# Autodesk Inventor assembly: linkage_system_test
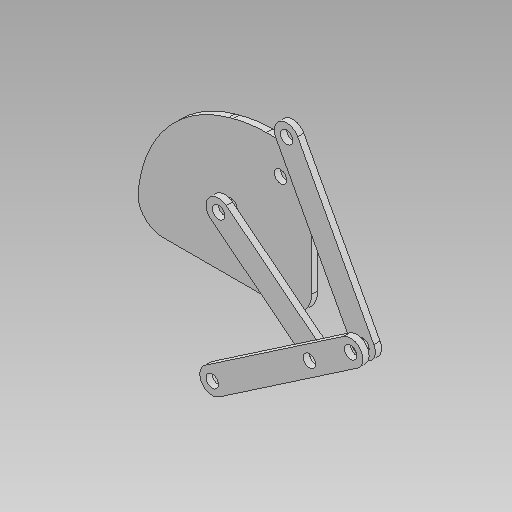
[picture p0: Inventor's stored thumbnail of the model, 512x512]
Saved by Autodesk Inventor 2025 (Build 290162000, 162)
## iProperties
Created: 2024-09-22
Part Number: linkage_system_test
Document SubType Name: Assembly
Designer: OSB
Title: S500 Frame
Author: OSB
Sending System: Autodesk Inventor 2021
Preprocessor: unknown
Minimum Resolution: 0.01
Sent Units: Millimeter
Translation Standard: IGES 5.3
Model Creation Time: 2020-07-07
## Documents named in this file (5)
- C:\Users\OSB\Desktop\SB\1.Projects\4_2\캡스톤 디자인(2)\linkage_system_test.iam
- C:\Users\OSB\Desktop\SB\1.Projects\4_2\캡스톤 디자인(2)\link_l1.ipt
- C:\Users\OSB\Desktop\SB\1.Projects\4_2\캡스톤 디자인(2)\link_l2.ipt
- C:\Users\OSB\Desktop\SB\1.Projects\4_2\캡스톤 디자인(2)\base.ipt
- C:\Users\OSB\Desktop\SB\1.Projects\4_2\캡스톤 디자인(2)\link_l34.ipt
## Components (4 placed, 4 different names)
1. link_l1:1 — 메이트:1, 메이트:2, 메이트:3, 메이트:4, 메이트:8, 메이트:9
2. link_l2:1 — 메이트:3, 메이트:5, 메이트:6, 메이트:7
3. base:1 — 메이트:4, 각도:1, 메이트:5, 메이트:6
4. link_l34:1 — 메이트:7, 메이트:8, 메이트:9
## Relationships (10: Mate 9, Angle 1)
- 메이트:1 [Mate]: link_l1:1
- 메이트:2 [Mate]: link_l1:1
- 메이트:3 [Mate]: link_l1:1 ↔ link_l2:1
- 메이트:4 [Mate]: link_l1:1 ↔ base:1
- 각도:1 [Angle] (0 deg): base:1
- 메이트:5 [Mate]: link_l2:1 ↔ base:1
- 메이트:6 [Mate]: link_l2:1 ↔ base:1
- 메이트:7 [Mate]: link_l2:1 ↔ link_l34:1
- 메이트:8 [Mate]: link_l1:1 ↔ link_l34:1
- 메이트:9 [Mate]: link_l1:1 ↔ link_l34:1
